# Autodesk Inventor assembly: vpol_hpol_cap_comparison
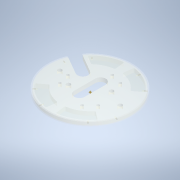
[picture p0: Inventor's stored thumbnail of the model, 180x180]
Saved by Autodesk Inventor 2021 (Build 250183000, 183)
## iProperties
Created: 2020-11-18
Part Number: vpol_hpol_cap_comparison
Document SubType Name: Assembly
Designer: dsouthall
Author: dsouthall
## Documents named in this file (3)
- C:\Users\dsouthall\OneDrive - The University of Chicago\Hpol\hpol-prototype\design\Quad-Slot\vpol_hpol_cap_comparison.iam
- C:\Users\dsouthall\OneDrive - The University of Chicago\Hpol\hpol-prototype\design\Vpol Parts\End Caps\hub_support.ipt
- C:\Users\dsouthall\OneDrive - The University of Chicago\Hpol\hpol-prototype\design\Quad-Slot\Model 8 in\source\End Cap.ipt
## Components (2 placed, 2 different names)
1. hub_support:1 — Mate:1, Mate:2
2. End Cap:1 — Mate:1, Mate:2
## Relationships (2: Mate 2)
- Mate:1: hub_support:1 ↔ End Cap:1
- Mate:2: hub_support:1 ↔ End Cap:1
